# Autodesk Inventor assembly: Pancake_Reverse Assy
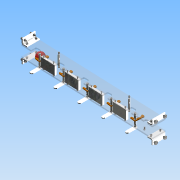
[picture p0: Inventor's stored thumbnail of the model, 180x180]
Saved by Autodesk Inventor 2018.1 (Build 221171000, 171)
## iProperties
Created: 2019-02-11
Part Number: Pancake_Reverse Assy
Document SubType Name: Assembly
Designer: James
Author: James
## Documents named in this file (20)
- C:\Users\admin\Desktop\Ball Sorting Machine\Ball-Sorting-Machine\Pancake Sort\Pancake_Reverse Assy.iam
- C:\Users\admin\Desktop\Ball Sorting Machine\Ball-Sorting-Machine\Pancake Sort\Nyloc Nut - M4.ipt
- C:\Users\admin\Desktop\Ball Sorting Machine\Ball-Sorting-Machine\Pancake Sort\Socket Cap Screw - Standard - (A2) - M4 x 16.ipt
- C:\Users\admin\Desktop\Ball Sorting Machine\Ball-Sorting-Machine\Pancake Sort\Pancake_Angle Bracket.ipt
- C:\Users\admin\Desktop\Ball Sorting Machine\Ball-Sorting-Machine\Selection Sort\Ball 30mm.ipt
- C:\Users\admin\Desktop\Ball Sorting Machine\Ball-Sorting-Machine\Pancake Sort\Pancake_Reverse Backboard 2.ipt
- C:\Users\admin\Desktop\Ball Sorting Machine\Ball-Sorting-Machine\Pancake Sort\Socket Csk Screw - (A2) - M4 x  12.ipt
- C:\Users\admin\Desktop\Ball Sorting Machine\Ball-Sorting-Machine\Pancake Sort\Pancake_Connector.ipt
- C:\Users\admin\Desktop\Ball Sorting Machine\Ball-Sorting-Machine\Pancake Sort\Socket Cap Screw - Standard - (A2) - M3 x 12.ipt
- C:\Users\admin\Desktop\Ball Sorting Machine\Ball-Sorting-Machine\Pancake Sort\Pancake_Bearing.ipt
- C:\Users\admin\Desktop\Ball Sorting Machine\Ball-Sorting-Machine\Pancake Sort\Pancake_Reverse Shaft.ipt
- C:\Users\admin\Desktop\Ball Sorting Machine\Ball-Sorting-Machine\Pancake Sort\Pancake_Reverse Lever.ipt
- C:\Users\admin\Desktop\Ball Sorting Machine\Ball-Sorting-Machine\Pancake Sort\BS 3673 - 6mm External Circlip.ipt
- C:\Users\admin\Desktop\Ball Sorting Machine\Ball-Sorting-Machine\Pancake Sort\Pancake_Reverse Weight.ipt
- C:\Users\admin\Desktop\Ball Sorting Machine\Ball-Sorting-Machine\Pancake Sort\Pancake_Reverse Backboard.ipt
- C:\Users\admin\Desktop\Ball Sorting Machine\Ball-Sorting-Machine\Pancake Sort\Locknut - M3.ipt
- C:\Users\admin\Desktop\Ball Sorting Machine\Ball-Sorting-Machine\Pancake Sort\Socket Csk Screw - (A2) - M3 x  10.ipt
- C:\Users\admin\Desktop\Ball Sorting Machine\Ball-Sorting-Machine\Pancake Sort\Pancake_Floor Piece.ipt
- C:\Users\admin\Desktop\Ball Sorting Machine\Ball-Sorting-Machine\Pancake Sort\Socket Csk Screw - (A2) - M4 x  16.ipt
- C:\Users\admin\Desktop\Ball Sorting Machine\Ball-Sorting-Machine\Pancake Sort\FWSRS-D12-V4.5-E2.5-T3_.ipt
## Components (109 placed, 19 different names)
1. Pancake_Reverse Backboard 2:1 — Mate:104, Mate:105, Mate:106, Flush:36, Mate:115, Flush:37, Mate:118, Mate:119, Mate:132, Tangent:2, Mate:138, Tangent:3, Mate:140, Mate:141, Tangent:4, Tangent:5, Mate:144, Flush:104, Flush:105, Mate:176, Mate:177, Mate:179, Mate:180, Mate:181, Mate:182, Mate:183, Mate:188, Mate:189, Flush:110, Flush:111, Mate:192, Mate:200, Mate:201, Mate:202, Mate:203, Mate:204, Tangent:15, Tangent:16
2. Pancake_Angle Bracket:3 — Mate:104, Mate:105, Mate:106, Flush:36, Mate:127, Mate:134, Mate:139, Mate:229, Mate:230
3. Pancake_Angle Bracket:4 — Mate:115, Flush:37, Mate:118, Mate:119, Mate:131, Mate:142, Mate:143, Mate:235, Mate:236, Mate:237
4. Pancake_Reverse Backboard:1 — Mate:144, Flush:104, Flush:105, Mate:155, Mate:156, Mate:157, Mate:158, Mate:159, Tangent:6, Tangent:7, Mate:170, Mate:171, Mate:173, Mate:174, Tangent:8, Tangent:9, Mate:175, Mate:178, Mate:184, Mate:185, Mate:186, Mate:187, Mate:190, Flush:112, Flush:113, Tangent:11, Mate:197, Tangent:12, Mate:198, Mate:205, Mate:206, Mate:207, Mate:208, Tangent:13, Tangent:14
5. Pancake_Angle Bracket:5 — Mate:155, Mate:156, Mate:157, Mate:226, Mate:227, Mate:228
6. Pancake_Angle Bracket:6 — Mate:170, Mate:171, Mate:175, Mate:238, Mate:239
7. Pancake_Connector:1 — Mate:176, Mate:177, Mate:178
8. Pancake_Connector:2 — Mate:179, Mate:180
9. Ball 30mm:1 — Tangent:10, Tangent:11
10. Socket Csk Screw - (A2) - M4 x  16:5 — Mate:236, Mate:242
11. FWSRS-D12-V4.5-E2.5-T3.0:5 — Flush:119, Mate:235
12. Socket Csk Screw - (A2) - M4 x  16:6 — Mate:237, Mate:243
13. FWSRS-D12-V4.5-E2.5-T3.0:6 — Flush:119, Flush:120
14. Socket Csk Screw - (A2) - M4 x  16:7 — Mate:238, Mate:240
15. FWSRS-D12-V4.5-E2.5-T3.0:7 — Flush:120, Flush:121
16. Socket Csk Screw - (A2) - M4 x  16:8 — Mate:239, Mate:241
17. FWSRS-D12-V4.5-E2.5-T3.0:8 — Flush:121
18. Socket Cap Screw - Standard - (A2) - M4 x 16:19 — Flush:116, Mate:226, Mate:227, Mate:233
19. Socket Cap Screw - Standard - (A2) - M4 x 16:20 — Flush:116, Flush:117, Mate:228, Mate:234
20. Socket Cap Screw - Standard - (A2) - M4 x 16:21 — Flush:117, Flush:118, Mate:229, Mate:232
21. Socket Cap Screw - Standard - (A2) - M4 x 16:22 — Flush:118, Mate:230, Mate:231
22. Nyloc Nut - M4:37 — Flush:99, Mate:127, Mate:231
23. Nyloc Nut - M4:38 — Flush:99, Mate:232
24. Nyloc Nut - M4:39 — Flush:101, Mate:131, Mate:242
25. Nyloc Nut - M4:40 — Flush:101, Mate:243
26. Socket Csk Screw - (A2) - M4 x  12:1 — Mate:132, Tangent:2, Mate:133
27. Nyloc Nut - M4:41 — Mate:133, Mate:134
28. Socket Csk Screw - (A2) - M4 x  12:2 — Mate:138, Tangent:3
29. Nyloc Nut - M4:42 — Mate:139
30. Socket Csk Screw - (A2) - M4 x  12:3 — Mate:141, Tangent:4
31. Nyloc Nut - M4:43 — Mate:142
32. Socket Csk Screw - (A2) - M4 x  12:4 — Mate:140, Tangent:5
33. Nyloc Nut - M4:44 — Mate:143
34. Nyloc Nut - M4:45 — Mate:234
35. Nyloc Nut - M4:46 — Mate:233
36. Socket Csk Screw - (A2) - M4 x  12:5 — Mate:158, Tangent:6
37. Nyloc Nut - M4:47
38. Socket Csk Screw - (A2) - M4 x  12:6 — Mate:159, Tangent:7
39. Nyloc Nut - M4:48
40. Nyloc Nut - M4:49 — Mate:240
41. Nyloc Nut - M4:50 — Mate:241
42. Socket Csk Screw - (A2) - M4 x  12:7 — Mate:173, Tangent:8
43. Nyloc Nut - M4:51
44. Socket Csk Screw - (A2) - M4 x  12:8 — Mate:174, Tangent:9
45. Nyloc Nut - M4:52
46. Socket Cap Screw - Standard - (A2) - M3 x 12:1 — Mate:181, Mate:182
47. Socket Cap Screw - Standard - (A2) - M3 x 12:2 — Mate:183, Mate:188
48. Socket Cap Screw - Standard - (A2) - M3 x 12:3 — Mate:184, Mate:187
49. Socket Cap Screw - Standard - (A2) - M3 x 12:4 — Mate:185, Mate:186
50. BS 3673 - 6mm External Circlip:1 — Mate:194, Mate:195, Angle:1
51. Pancake_Reverse Lever:1 — Mate:193, Flush:114, Angle:1, Angle:2, Tangent:10
52. Pancake_Reverse Shaft:1 — Mate:191, Mate:192, Mate:193, Flush:114, Mate:194, Mate:195, Mate:196, Flush:115
53. Pancake_Bearing:1 — Mate:189, Flush:110, Flush:111, Mate:191
54. Pancake_Reverse Weight:1 — Mate:196, Flush:115, Angle:2
55. Pancake_Bearing:2 — Mate:190, Flush:112, Flush:113
56. BS 3673 - 6mm External Circlip:2
57. Pancake_Reverse Lever:2
58. Pancake_Reverse Shaft:2
59. Pancake_Bearing:3
60. Pancake_Reverse Weight:2
61. Pancake_Bearing:4
62. BS 3673 - 6mm External Circlip:3
63. Pancake_Reverse Lever:3
64. Pancake_Reverse Shaft:3
65. Pancake_Bearing:5
66. Pancake_Reverse Weight:3
67. Pancake_Bearing:6
68. BS 3673 - 6mm External Circlip:4
69. Pancake_Reverse Lever:4
70. Pancake_Reverse Shaft:4
71. Pancake_Bearing:7
72. Pancake_Reverse Weight:4
73. Pancake_Bearing:8
74. BS 3673 - 6mm External Circlip:5
75. Pancake_Reverse Lever:5
76. Pancake_Reverse Shaft:5
77. Pancake_Bearing:9
78. Pancake_Reverse Weight:5
79. Pancake_Bearing:10
80. Socket Csk Screw - (A2) - M3 x  10:1 — Mate:197, Tangent:12, Mate:199
81. Locknut - M3:1 — Mate:198, Mate:199
82. Socket Csk Screw - (A2) - M3 x  10:2
83. Locknut - M3:2
84. Socket Csk Screw - (A2) - M3 x  10:3
85. Locknut - M3:3
86. Socket Csk Screw - (A2) - M3 x  10:4
87. Locknut - M3:4
88. Socket Csk Screw - (A2) - M3 x  10:5
89. Locknut - M3:5
90. Pancake_Floor Piece:1 — Mate:200, Mate:201, Mate:202, Mate:207, Mate:208
91. Socket Csk Screw - (A2) - M3 x  10:9 — Mate:205, Tangent:13
92. Socket Csk Screw - (A2) - M3 x  10:8 — Mate:203, Tangent:15
93. Socket Csk Screw - (A2) - M3 x  10:7 — Mate:206, Tangent:14
94. Socket Csk Screw - (A2) - M3 x  10:6 — Mate:204, Tangent:16
95. Pancake_Floor Piece:2
96. Socket Csk Screw - (A2) - M3 x  10:10
97. Socket Csk Screw - (A2) - M3 x  10:11
98. Socket Csk Screw - (A2) - M3 x  10:12
99. Socket Csk Screw - (A2) - M3 x  10:13
100. Pancake_Floor Piece:3
101. Socket Csk Screw - (A2) - M3 x  10:14
102. Socket Csk Screw - (A2) - M3 x  10:15
103. Socket Csk Screw - (A2) - M3 x  10:16
104. Socket Csk Screw - (A2) - M3 x  10:17
105. Pancake_Floor Piece:4
106. Socket Csk Screw - (A2) - M3 x  10:18
107. Socket Csk Screw - (A2) - M3 x  10:19
108. Socket Csk Screw - (A2) - M3 x  10:20
109. Socket Csk Screw - (A2) - M3 x  10:21
## Component patterns: (5 elements, first: BS 3673 - 6mm External Circlip:1 + Pancake_Reverse Lever:1 + Pancake_Reverse Shaft:1 + Pancake_Bearing:1 + Pancake_Reverse Weight:1 + Pancake_Bearing:2), (5 elements, first: Socket Csk Screw - (A2) - M3 x  10:1 + Locknut - M3:1), (4 elements, first: Pancake_Floor Piece:1 + Socket Csk Screw - (A2) - M3 x  10:9 + Socket Csk Screw - (A2) - M3 x  10:8 + Socket Csk Screw - (A2) - M3 x  10:7 + Socket Csk Screw - (A2) - M3 x  10:6)
## Relationships (142: Mate 96, Flush 25, Tangent 19, Angle 2)
- Flush:11 (62.5 mm)
- [Flush]: Pancake_Reverse Backboard 2:1
- [Flush]: Pancake_Reverse Backboard 2:1
- [Flush]: Pancake_Reverse Backboard 2:1
- Mate:104: Pancake_Reverse Backboard 2:1 ↔ Pancake_Angle Bracket:3
- Mate:105: Pancake_Reverse Backboard 2:1 ↔ Pancake_Angle Bracket:3
- Mate:106: Pancake_Reverse Backboard 2:1 ↔ Pancake_Angle Bracket:3
- Flush:36: Pancake_Reverse Backboard 2:1 ↔ Pancake_Angle Bracket:3
- Mate:115: Pancake_Reverse Backboard 2:1 ↔ Pancake_Angle Bracket:4
- Flush:37: Pancake_Reverse Backboard 2:1 ↔ Pancake_Angle Bracket:4
- Mate:118: Pancake_Reverse Backboard 2:1 ↔ Pancake_Angle Bracket:4
- Mate:119: Pancake_Reverse Backboard 2:1 ↔ Pancake_Angle Bracket:4
- Flush:99: Nyloc Nut - M4:37 ↔ Nyloc Nut - M4:38
- Mate:127: Pancake_Angle Bracket:3 ↔ Nyloc Nut - M4:37
- Flush:101: Nyloc Nut - M4:39 ↔ Nyloc Nut - M4:40
- Mate:131: Pancake_Angle Bracket:4 ↔ Nyloc Nut - M4:39
- Flush:103 (35 mm)
- Mate:132: Pancake_Reverse Backboard 2:1 ↔ Socket Csk Screw - (A2) - M4 x  12:1
- Tangent:2: Pancake_Reverse Backboard 2:1 ↔ Socket Csk Screw - (A2) - M4 x  12:1
- Mate:133: Socket Csk Screw - (A2) - M4 x  12:1 ↔ Nyloc Nut - M4:41
- Mate:134: Pancake_Angle Bracket:3 ↔ Nyloc Nut - M4:41
- [Mate]: Socket Csk Screw - (A2) - M4 x  12:2 ↔ Nyloc Nut - M4:42
- [Mate]: Socket Csk Screw - (A2) - M4 x  12:3 ↔ Nyloc Nut - M4:43
- [Mate]: Socket Csk Screw - (A2) - M4 x  12:4 ↔ Nyloc Nut - M4:44
- Mate:138: Pancake_Reverse Backboard 2:1 ↔ Socket Csk Screw - (A2) - M4 x  12:2
- Tangent:3: Pancake_Reverse Backboard 2:1 ↔ Socket Csk Screw - (A2) - M4 x  12:2
- Mate:139: Pancake_Angle Bracket:3 ↔ Nyloc Nut - M4:42
- Mate:140: Pancake_Reverse Backboard 2:1 ↔ Socket Csk Screw - (A2) - M4 x  12:4
- Mate:141: Pancake_Reverse Backboard 2:1 ↔ Socket Csk Screw - (A2) - M4 x  12:3
- Tangent:4: Pancake_Reverse Backboard 2:1 ↔ Socket Csk Screw - (A2) - M4 x  12:3
- Tangent:5: Pancake_Reverse Backboard 2:1 ↔ Socket Csk Screw - (A2) - M4 x  12:4
- Mate:142: Pancake_Angle Bracket:4 ↔ Nyloc Nut - M4:43
- Mate:143: Pancake_Angle Bracket:4 ↔ Nyloc Nut - M4:44
- Mate:144 (35 mm): Pancake_Reverse Backboard 2:1 ↔ Pancake_Reverse Backboard:1
- Flush:104: Pancake_Reverse Backboard 2:1 ↔ Pancake_Reverse Backboard:1
- Flush:105: Pancake_Reverse Backboard 2:1 ↔ Pancake_Reverse Backboard:1
- [Flush]: Nyloc Nut - M4:45 ↔ Nyloc Nut - M4:46
- [Mate]: Pancake_Angle Bracket:5 ↔ Nyloc Nut - M4:45
- [Mate]: Socket Csk Screw - (A2) - M4 x  12:5 ↔ Nyloc Nut - M4:47
- [Mate]: Pancake_Angle Bracket:5 ↔ Nyloc Nut - M4:47
- [Mate]: Socket Csk Screw - (A2) - M4 x  12:6 ↔ Nyloc Nut - M4:48
- [Mate]: Pancake_Angle Bracket:5 ↔ Nyloc Nut - M4:48
- Mate:155: Pancake_Reverse Backboard:1 ↔ Pancake_Angle Bracket:5
- Mate:156: Pancake_Reverse Backboard:1 ↔ Pancake_Angle Bracket:5
- Mate:157: Pancake_Reverse Backboard:1 ↔ Pancake_Angle Bracket:5
- Mate:158: Pancake_Reverse Backboard:1 ↔ Socket Csk Screw - (A2) - M4 x  12:5
- Mate:159: Pancake_Reverse Backboard:1 ↔ Socket Csk Screw - (A2) - M4 x  12:6
- Tangent:6: Pancake_Reverse Backboard:1 ↔ Socket Csk Screw - (A2) - M4 x  12:5
- Tangent:7: Pancake_Reverse Backboard:1 ↔ Socket Csk Screw - (A2) - M4 x  12:6
- [Flush]: Nyloc Nut - M4:49 ↔ Nyloc Nut - M4:50
- [Mate]: Pancake_Angle Bracket:6 ↔ Nyloc Nut - M4:49
- [Mate]: Socket Csk Screw - (A2) - M4 x  12:7 ↔ Nyloc Nut - M4:51
- [Mate]: Pancake_Angle Bracket:6 ↔ Nyloc Nut - M4:51
- [Mate]: Socket Csk Screw - (A2) - M4 x  12:8 ↔ Nyloc Nut - M4:52
- [Mate]: Pancake_Angle Bracket:6 ↔ Nyloc Nut - M4:52
- Mate:170: Pancake_Reverse Backboard:1 ↔ Pancake_Angle Bracket:6
- Mate:171: Pancake_Reverse Backboard:1 ↔ Pancake_Angle Bracket:6
- Mate:173: Pancake_Reverse Backboard:1 ↔ Socket Csk Screw - (A2) - M4 x  12:7
- Mate:174: Pancake_Reverse Backboard:1 ↔ Socket Csk Screw - (A2) - M4 x  12:8
- Tangent:8: Pancake_Reverse Backboard:1 ↔ Socket Csk Screw - (A2) - M4 x  12:7
- Tangent:9: Pancake_Reverse Backboard:1 ↔ Socket Csk Screw - (A2) - M4 x  12:8
- Mate:175: Pancake_Reverse Backboard:1 ↔ Pancake_Angle Bracket:6
- Mate:176: Pancake_Reverse Backboard 2:1 ↔ Pancake_Connector:1
- Mate:177: Pancake_Reverse Backboard 2:1 ↔ Pancake_Connector:1
- Mate:178: Pancake_Reverse Backboard:1 ↔ Pancake_Connector:1
- Mate:179: Pancake_Reverse Backboard 2:1 ↔ Pancake_Connector:2
- Mate:180: Pancake_Reverse Backboard 2:1 ↔ Pancake_Connector:2
- Mate:181: Pancake_Reverse Backboard 2:1 ↔ Socket Cap Screw - Standard - (A2) - M3 x 12:1
- Mate:182: Pancake_Reverse Backboard 2:1 ↔ Socket Cap Screw - Standard - (A2) - M3 x 12:1
- Mate:183: Pancake_Reverse Backboard 2:1 ↔ Socket Cap Screw - Standard - (A2) - M3 x 12:2
- Mate:184: Pancake_Reverse Backboard:1 ↔ Socket Cap Screw - Standard - (A2) - M3 x 12:3
- Mate:185: Pancake_Reverse Backboard:1 ↔ Socket Cap Screw - Standard - (A2) - M3 x 12:4
- Mate:186: Pancake_Reverse Backboard:1 ↔ Socket Cap Screw - Standard - (A2) - M3 x 12:4
- Mate:187: Pancake_Reverse Backboard:1 ↔ Socket Cap Screw - Standard - (A2) - M3 x 12:3
- Mate:188: Pancake_Reverse Backboard 2:1 ↔ Socket Cap Screw - Standard - (A2) - M3 x 12:2
- Mate:189: Pancake_Reverse Backboard 2:1 ↔ Pancake_Bearing:1
- Flush:110: Pancake_Reverse Backboard 2:1 ↔ Pancake_Bearing:1
- Flush:111: Pancake_Reverse Backboard 2:1 ↔ Pancake_Bearing:1
- Mate:190: Pancake_Reverse Backboard:1 ↔ Pancake_Bearing:2
- Flush:112: Pancake_Reverse Backboard:1 ↔ Pancake_Bearing:2
- Flush:113: Pancake_Reverse Backboard:1 ↔ Pancake_Bearing:2
- Mate:191: Pancake_Reverse Shaft:1 ↔ Pancake_Bearing:1
- Mate:192 (0.5 mm): Pancake_Reverse Backboard 2:1 ↔ Pancake_Reverse Shaft:1
- Mate:193: Pancake_Reverse Lever:1 ↔ Pancake_Reverse Shaft:1
- Flush:114: Pancake_Reverse Lever:1 ↔ Pancake_Reverse Shaft:1
- Mate:194: BS 3673 - 6mm External Circlip:1 ↔ Pancake_Reverse Shaft:1
- Mate:195: BS 3673 - 6mm External Circlip:1 ↔ Pancake_Reverse Shaft:1
- Angle:1 (0 deg): BS 3673 - 6mm External Circlip:1 ↔ Pancake_Reverse Lever:1
- Mate:196: Pancake_Reverse Shaft:1 ↔ Pancake_Reverse Weight:1
- Flush:115 (-0.5 mm): Pancake_Reverse Shaft:1 ↔ Pancake_Reverse Weight:1
- Angle:2 (5 deg): Pancake_Reverse Lever:1 ↔ Pancake_Reverse Weight:1
- Tangent:10: Ball 30mm:1 ↔ Pancake_Reverse Lever:1
- Tangent:11: Pancake_Reverse Backboard:1 ↔ Ball 30mm:1
- Mate:197: Pancake_Reverse Backboard:1 ↔ Socket Csk Screw - (A2) - M3 x  10:1
- Tangent:12: Pancake_Reverse Backboard:1 ↔ Socket Csk Screw - (A2) - M3 x  10:1
- Mate:198: Pancake_Reverse Backboard:1 ↔ Locknut - M3:1
- Mate:199: Socket Csk Screw - (A2) - M3 x  10:1 ↔ Locknut - M3:1
- Mate:200: Pancake_Reverse Backboard 2:1 ↔ Pancake_Floor Piece:1
- Mate:201: Pancake_Reverse Backboard 2:1 ↔ Pancake_Floor Piece:1
- Mate:202: Pancake_Reverse Backboard 2:1 ↔ Pancake_Floor Piece:1
- Mate:203: Pancake_Reverse Backboard 2:1 ↔ Socket Csk Screw - (A2) - M3 x  10:8
- Mate:204: Pancake_Reverse Backboard 2:1 ↔ Socket Csk Screw - (A2) - M3 x  10:6
- Mate:205: Pancake_Reverse Backboard:1 ↔ Socket Csk Screw - (A2) - M3 x  10:9
- Mate:206: Pancake_Reverse Backboard:1 ↔ Socket Csk Screw - (A2) - M3 x  10:7
- Mate:207: Pancake_Reverse Backboard:1 ↔ Pancake_Floor Piece:1
- Mate:208: Pancake_Reverse Backboard:1 ↔ Pancake_Floor Piece:1
- Tangent:13: Pancake_Reverse Backboard:1 ↔ Socket Csk Screw - (A2) - M3 x  10:9
- Tangent:14: Pancake_Reverse Backboard:1 ↔ Socket Csk Screw - (A2) - M3 x  10:7
- Tangent:15: Pancake_Reverse Backboard 2:1 ↔ Socket Csk Screw - (A2) - M3 x  10:8
- Tangent:16: Pancake_Reverse Backboard 2:1 ↔ Socket Csk Screw - (A2) - M3 x  10:6
- [Mate]: Socket Csk Screw - (A2) - M4 x  16:5 ↔ FWSRS-D12-V4.5-E2.5-T3.0:5
- [Tangent]: Socket Csk Screw - (A2) - M4 x  16:5 ↔ FWSRS-D12-V4.5-E2.5-T3.0:5
- [Mate]: Socket Csk Screw - (A2) - M4 x  16:6 ↔ FWSRS-D12-V4.5-E2.5-T3.0:6
- [Tangent]: Socket Csk Screw - (A2) - M4 x  16:6 ↔ FWSRS-D12-V4.5-E2.5-T3.0:6
- [Mate]: Socket Csk Screw - (A2) - M4 x  16:7 ↔ FWSRS-D12-V4.5-E2.5-T3.0:7
- [Tangent]: Socket Csk Screw - (A2) - M4 x  16:7 ↔ FWSRS-D12-V4.5-E2.5-T3.0:7
- [Mate]: Socket Csk Screw - (A2) - M4 x  16:8 ↔ FWSRS-D12-V4.5-E2.5-T3.0:8
- [Tangent]: Socket Csk Screw - (A2) - M4 x  16:8 ↔ FWSRS-D12-V4.5-E2.5-T3.0:8
- Flush:116: Socket Cap Screw - Standard - (A2) - M4 x 16:19 ↔ Socket Cap Screw - Standard - (A2) - M4 x 16:20
- Flush:117: Socket Cap Screw - Standard - (A2) - M4 x 16:20 ↔ Socket Cap Screw - Standard - (A2) - M4 x 16:21
- Flush:118: Socket Cap Screw - Standard - (A2) - M4 x 16:21 ↔ Socket Cap Screw - Standard - (A2) - M4 x 16:22
- Mate:226 (5 mm): Pancake_Angle Bracket:5 ↔ Socket Cap Screw - Standard - (A2) - M4 x 16:19
- Mate:227: Pancake_Angle Bracket:5 ↔ Socket Cap Screw - Standard - (A2) - M4 x 16:19
- Mate:228: Pancake_Angle Bracket:5 ↔ Socket Cap Screw - Standard - (A2) - M4 x 16:20
- Mate:229: Pancake_Angle Bracket:3 ↔ Socket Cap Screw - Standard - (A2) - M4 x 16:21
- Mate:230: Pancake_Angle Bracket:3 ↔ Socket Cap Screw - Standard - (A2) - M4 x 16:22
- Mate:231: Socket Cap Screw - Standard - (A2) - M4 x 16:22 ↔ Nyloc Nut - M4:37
- Mate:232: Socket Cap Screw - Standard - (A2) - M4 x 16:21 ↔ Nyloc Nut - M4:38
- Mate:233: Socket Cap Screw - Standard - (A2) - M4 x 16:19 ↔ Nyloc Nut - M4:46
- Mate:234: Socket Cap Screw - Standard - (A2) - M4 x 16:20 ↔ Nyloc Nut - M4:45
- Flush:119: FWSRS-D12-V4.5-E2.5-T3.0:5 ↔ FWSRS-D12-V4.5-E2.5-T3.0:6
- Flush:120: FWSRS-D12-V4.5-E2.5-T3.0:6 ↔ FWSRS-D12-V4.5-E2.5-T3.0:7
- Flush:121: FWSRS-D12-V4.5-E2.5-T3.0:7 ↔ FWSRS-D12-V4.5-E2.5-T3.0:8
- Mate:235 (5 mm): Pancake_Angle Bracket:4 ↔ FWSRS-D12-V4.5-E2.5-T3.0:5
- Mate:236: Pancake_Angle Bracket:4 ↔ Socket Csk Screw - (A2) - M4 x  16:5
- Mate:237: Pancake_Angle Bracket:4 ↔ Socket Csk Screw - (A2) - M4 x  16:6
- Mate:238: Pancake_Angle Bracket:6 ↔ Socket Csk Screw - (A2) - M4 x  16:7
- Mate:239: Pancake_Angle Bracket:6 ↔ Socket Csk Screw - (A2) - M4 x  16:8
- Mate:240: Socket Csk Screw - (A2) - M4 x  16:7 ↔ Nyloc Nut - M4:49
- Mate:241: Socket Csk Screw - (A2) - M4 x  16:8 ↔ Nyloc Nut - M4:50
- Mate:242: Socket Csk Screw - (A2) - M4 x  16:5 ↔ Nyloc Nut - M4:39
- Mate:243: Socket Csk Screw - (A2) - M4 x  16:6 ↔ Nyloc Nut - M4:40
## Named parameters: d253_d251 = 0 mm, d254_d251 = 0 mm, d255_d251 = 0 mm, d268_d251 = 0 mm, d269_d252 = 0 mm, d270_d253_d251 = 0 mm, d271_d258 = 0 mm, d276_d219 = 0 mm, d277_d220 = 0 mm, d287_d251 = 0 mm, d288_d252 = 0 mm, d289_d253_d251 = 0 mm, d290_d258 = 0 mm, d295_d219 = 0 mm, d296_d220 = 0 mm, d398_d387 = 0 mm, d399_d388 = 0 mm, d400_d387 = 0 mm, d401_d388 = 0 mm, d402_d387 = 0 mm, d403_d388 = 0 mm, d404_d387 = 0 mm, d405_d388 = 0 mm
